# Autodesk Inventor assembly: Finished Lamp
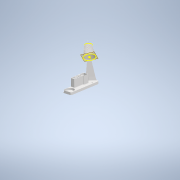
[picture p0: Inventor's stored thumbnail of the model, 180x180]
Saved by Autodesk Inventor 2020 (Build 240168000, 168)
## iProperties
Created: 2020-09-14
Part Number: Finished Lamp
Document SubType Name: Assembly
Designer: samhita001
Author: samhita001
## Documents named in this file (6)
- C:\Users\samhi\Downloads\Lamp Final\Lamp\Finished Lamp.iam
- C:\Users\samhi\Downloads\Lamp Final\Lamp\Lamp Parts\LampBase.ipt
- C:\Users\samhi\Downloads\Lamp Final\Lamp\Lamp Parts\Lampshade.ipt
- C:\Users\samhi\Downloads\Lamp Final\Lamp\Lamp Parts\bulbbase.ipt
- C:\Users\samhi\Downloads\Lamp Final\Lamp\Lamp Parts\miniscrew.ipt
- C:\Users\samhi\Downloads\Lamp Final\Lamp\Lamp Parts\bulbholder.ipt
## Components (5 placed, 5 different names)
1. LampBase:1 — Mate:2, Mate:3, Mate:4
2. Lampshade:1 — Mate:2, Mate:3, Mate:5
3. bulbbase:1 — Mate:4, Mate:5, Mate:6, Mate:7
4. miniscrew:1 — Mate:6
5. bulbholder:1 — Mate:7
## Relationships (6: Mate 6)
- Mate:2: LampBase:1 ↔ Lampshade:1
- Mate:3: LampBase:1 ↔ Lampshade:1
- Mate:4: LampBase:1 ↔ bulbbase:1
- Mate:5: Lampshade:1 ↔ bulbbase:1
- Mate:6: bulbbase:1 ↔ miniscrew:1
- Mate:7: bulbbase:1 ↔ bulbholder:1
